# Autodesk Inventor assembly: map #2
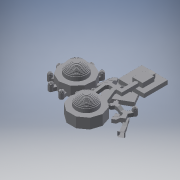
[picture p0: Inventor's stored thumbnail of the model, 180x180]
Saved by Autodesk Inventor 2017 (Build 210142000, 142)
## iProperties
Created: 2018-05-09
Part Number: map #2
Document SubType Name: Assembly
Designer: braxtonwright
Author: braxtonwright
## Documents named in this file (13)
- E:\School\Game develpment\geoscape\assembly\map #2.iam
- E:\School\Game develpment\geoscape\done\lowend map componts\corridors\corridor 2nd map.ipt
- E:\School\Game develpment\geoscape\done\lowend map componts\corridors\corridor 90 turn 2nd map.ipt
- E:\School\Game develpment\geoscape\done\lowend map componts\corridors\X corridor 2nd map.ipt
- E:\School\Game develpment\geoscape\done\lowend map componts\corridors\Y corridor 2nd map.ipt
- E:\School\Game develpment\geoscape\done\lowend map componts\rooms\starting room 2nd map.ipt
- E:\School\Game develpment\geoscape\done\lowend map componts\corridors\ramp 2nd map.ipt
- E:\School\Game develpment\geoscape\done\lowend map componts\rooms\room with 15 cubicals 2nd map.ipt
- E:\School\Game develpment\geoscape\done\lowend map componts\rooms\dome 2nd map.ipt
- E:\School\Game develpment\geoscape\done\lowend map componts\rooms\dome with corridors 2nd map.ipt
- E:\School\Game develpment\geoscape\done\lowend map componts\rooms\dome one terminal 2nd map.ipt
- E:\School\Game develpment\geoscape\rooms\(closed face) end door room (one wall) (9) 2nd map.ipt
- E:\School\Game develpment\geoscape\rooms\end door room (one wall) (9) 2nd map.ipt
## Components (56 placed, 12 different names)
1. corridor 2nd map:3 — Mate:91, Mate:92, Mate:97, Mate:98
2. ramp 2nd map:24 — Mate:89, Mate:90, Mate:91, Mate:92
3. ramp 2nd map:23 — Mate:85, Mate:86, Mate:87, Mate:88
4. ramp 2nd map:22 — Mate:81, Mate:82, Mate:83, Mate:84
5. ramp 2nd map:21 — Mate:77, Mate:78, Mate:79, Mate:80
6. corridor 90 turn 2nd map:9 — Mate:87, Mate:88, Mate:89, Mate:90
7. corridor 90 turn 2nd map:8 — Mate:83, Mate:84, Mate:85, Mate:86
8. corridor 90 turn 2nd map:7 — Mate:79, Mate:80, Mate:81, Mate:82
9. corridor 90 turn 2nd map:6 — Mate:77, Mate:78, Mate:93, Mate:94
10. Y corridor 2nd map:3 — Mate:73, Mate:74, Mate:75, Mate:76, Mate:93, Mate:94
11. ramp 2nd map:20 — Mate:71, Mate:72, Mate:73, Mate:74
12. Y corridor 2nd map:2 — Mate:67, Mate:68, Mate:69, Mate:70, Mate:71, Mate:72
13. ramp 2nd map:19 — Mate:61, Mate:62, Mate:67, Mate:68
14. ramp 2nd map:18 — Mate:60, Mate:61, Mate:62, Mate:63
15. ramp 2nd map:17 — Mate:59, Mate:60, Mate:63, Mate:64
16. ramp 2nd map:16 — Mate:59, Mate:64, Mate:65, Mate:66
17. corridor 90 turn 2nd map:5 — Mate:57, Mate:58, Mate:65, Mate:66
18. corridor 90 turn 2nd map:4 — Mate:55, Mate:56, Mate:57, Mate:58
19. ramp 2nd map:15 — Mate:31, Mate:34, Mate:35, Mate:36
20. ramp 2nd map:14 — Mate:30, Mate:31, Mate:33, Mate:34
21. ramp 2nd map:13 — Mate:29, Mate:30, Mate:32, Mate:33
22. corridor 2nd map:1 — Flush:1, Flush:5, Mate:1, Mate:5, Mate:6
23. corridor 2nd map:2 — Flush:1, Flush:2, Flush:5, Flush:6, Mate:1, Mate:2
24. corridor 90 turn 2nd map:2 — Flush:2, Flush:3, Flush:6, Flush:7, Mate:2, Mate:3
25. X corridor 2nd map:1 — Flush:3, Flush:4, Flush:7, Flush:8, Mate:3, Mate:4, Mate:7, Mate:10, Mate:19, Mate:22
26. Y corridor 2nd map:1 — Flush:4, Flush:8, Mate:4, Mate:8, Mate:9, Mate:20, Mate:21
27. ramp 2nd map:1 — Mate:9, Flush:17, Mate:15, Mate:20
28. ramp 2nd map:2 — Flush:19, Flush:20, Mate:17, Mate:18
29. ramp 2nd map:3 — Flush:20, Mate:18, Mate:25, Mate:26
30. ramp 2nd map:4 — Mate:10, Flush:19, Mate:17, Mate:19
31. ramp 2nd map:5 — Flush:17, Flush:18, Mate:15, Mate:16
32. ramp 2nd map:6 — Flush:18, Mate:16, Mate:55, Mate:56
33. ramp 2nd map:7 — Mate:8, Flush:15, Mate:13, Mate:21
34. ramp 2nd map:8 — Flush:15, Flush:16, Mate:13, Mate:14
35. ramp 2nd map:9 — Flush:16, Mate:14, Mate:27, Mate:28, Mate:29
36. ramp 2nd map:10 — Mate:7, Flush:13, Mate:11, Mate:22
37. ramp 2nd map:11 — Flush:13, Flush:14, Mate:11, Mate:12
38. ramp 2nd map:12 — Flush:14, Mate:12, Mate:23, Mate:24
39. dome 2nd map:1 — Mate:25, Mate:26
40. corridor 90 turn 2nd map:3 — Mate:27, Mate:28, Mate:32
41. (closed face) end door room (one wall) (9) 2nd map:1 — Mate:95, Mate:96
42. end door room (one wall) (9) 2nd map:1 — Mate:97, Mate:98
43. dome one terminal 2nd map:10 — Mate:75, Mate:76
44. room with 15 cubicals 2nd map:2 — Mate:69, Mate:70
45. dome with corridors 2nd map:1 — Mate:35, Mate:36, Mate:37, Mate:38, Mate:39, Mate:40, Mate:41, Mate:42, Mate:43, Mate:44, Mate:45, Mate:46, Mate:47, Mate:48, Mate:49, Mate:50, Mate:51, Mate:52, Mate:53, Mate:54
46. dome one terminal 2nd map:1 — Mate:37, Mate:54
47. dome one terminal 2nd map:2 — Mate:38, Mate:46
48. dome one terminal 2nd map:3 — Mate:39, Mate:47
49. dome one terminal 2nd map:4 — Mate:40, Mate:48
50. dome one terminal 2nd map:5 — Mate:41, Mate:49
51. dome one terminal 2nd map:6 — Mate:42, Mate:50
52. dome one terminal 2nd map:7 — Mate:43, Mate:51
53. dome one terminal 2nd map:8 — Mate:44, Mate:52
54. dome one terminal 2nd map:9 — Mate:45, Mate:53
55. starting room 2nd map:1 — Mate:5, Mate:6, Mate:95, Mate:96
56. room with 15 cubicals 2nd map:1 — Mate:23, Mate:24
## Relationships (114: Mate 98, Flush 16)
- Flush:1: corridor 2nd map:1 ↔ corridor 2nd map:2
- Flush:2: corridor 2nd map:2 ↔ corridor 90 turn 2nd map:2
- Flush:3: corridor 90 turn 2nd map:2 ↔ X corridor 2nd map:1
- Flush:4: X corridor 2nd map:1 ↔ Y corridor 2nd map:1
- Flush:5: corridor 2nd map:1 ↔ corridor 2nd map:2
- Flush:6: corridor 2nd map:2 ↔ corridor 90 turn 2nd map:2
- Flush:7: corridor 90 turn 2nd map:2 ↔ X corridor 2nd map:1
- Flush:8: X corridor 2nd map:1 ↔ Y corridor 2nd map:1
- Mate:1: corridor 2nd map:1 ↔ corridor 2nd map:2
- Mate:2: corridor 2nd map:2 ↔ corridor 90 turn 2nd map:2
- Mate:3: corridor 90 turn 2nd map:2 ↔ X corridor 2nd map:1
- Mate:4: X corridor 2nd map:1 ↔ Y corridor 2nd map:1
- Mate:5: corridor 2nd map:1 ↔ starting room 2nd map:1
- Mate:6: corridor 2nd map:1 ↔ starting room 2nd map:1
- Mate:7: X corridor 2nd map:1 ↔ ramp 2nd map:10
- Mate:8: Y corridor 2nd map:1 ↔ ramp 2nd map:7
- Mate:9: Y corridor 2nd map:1 ↔ ramp 2nd map:1
- Mate:10: X corridor 2nd map:1 ↔ ramp 2nd map:4
- Flush:13: ramp 2nd map:10 ↔ ramp 2nd map:11
- Flush:14: ramp 2nd map:11 ↔ ramp 2nd map:12
- Mate:11: ramp 2nd map:10 ↔ ramp 2nd map:11
- Mate:12: ramp 2nd map:11 ↔ ramp 2nd map:12
- Flush:15: ramp 2nd map:7 ↔ ramp 2nd map:8
- Flush:16: ramp 2nd map:8 ↔ ramp 2nd map:9
- Mate:13: ramp 2nd map:7 ↔ ramp 2nd map:8
- Mate:14: ramp 2nd map:8 ↔ ramp 2nd map:9
- Flush:17: ramp 2nd map:1 ↔ ramp 2nd map:5
- Flush:18: ramp 2nd map:5 ↔ ramp 2nd map:6
- Mate:15: ramp 2nd map:1 ↔ ramp 2nd map:5
- Mate:16: ramp 2nd map:5 ↔ ramp 2nd map:6
- Flush:19: ramp 2nd map:2 ↔ ramp 2nd map:4
- Flush:20: ramp 2nd map:2 ↔ ramp 2nd map:3
- Mate:17: ramp 2nd map:2 ↔ ramp 2nd map:4
- Mate:18: ramp 2nd map:2 ↔ ramp 2nd map:3
- Mate:19: X corridor 2nd map:1 ↔ ramp 2nd map:4
- Mate:20: Y corridor 2nd map:1 ↔ ramp 2nd map:1
- Mate:21: Y corridor 2nd map:1 ↔ ramp 2nd map:7
- Mate:22: X corridor 2nd map:1 ↔ ramp 2nd map:10
- Mate:23: ramp 2nd map:12 ↔ room with 15 cubicals 2nd map:1
- Mate:24: ramp 2nd map:12 ↔ room with 15 cubicals 2nd map:1
- Mate:25: ramp 2nd map:3 ↔ dome 2nd map:1
- Mate:26: ramp 2nd map:3 ↔ dome 2nd map:1
- Mate:27: ramp 2nd map:9 ↔ corridor 90 turn 2nd map:3
- Mate:28: ramp 2nd map:9 ↔ corridor 90 turn 2nd map:3
- Mate:29: ramp 2nd map:13 ↔ ramp 2nd map:9
- Mate:30: ramp 2nd map:14 ↔ ramp 2nd map:13
- Mate:31: ramp 2nd map:15 ↔ ramp 2nd map:14
- Mate:32: ramp 2nd map:13 ↔ corridor 90 turn 2nd map:3
- Mate:33: ramp 2nd map:14 ↔ ramp 2nd map:13
- Mate:34: ramp 2nd map:15 ↔ ramp 2nd map:14
- Mate:35: ramp 2nd map:15 ↔ dome with corridors 2nd map:1
- Mate:36: ramp 2nd map:15 ↔ dome with corridors 2nd map:1
- Mate:37: dome with corridors 2nd map:1 ↔ dome one terminal 2nd map:1
- Mate:38: dome with corridors 2nd map:1 ↔ dome one terminal 2nd map:2
- Mate:39: dome with corridors 2nd map:1 ↔ dome one terminal 2nd map:3
- Mate:40: dome with corridors 2nd map:1 ↔ dome one terminal 2nd map:4
- Mate:41: dome with corridors 2nd map:1 ↔ dome one terminal 2nd map:5
- Mate:42: dome with corridors 2nd map:1 ↔ dome one terminal 2nd map:6
- Mate:43: dome with corridors 2nd map:1 ↔ dome one terminal 2nd map:7
- Mate:44: dome with corridors 2nd map:1 ↔ dome one terminal 2nd map:8
- Mate:45: dome with corridors 2nd map:1 ↔ dome one terminal 2nd map:9
- Mate:46: dome with corridors 2nd map:1 ↔ dome one terminal 2nd map:2
- Mate:47: dome with corridors 2nd map:1 ↔ dome one terminal 2nd map:3
- Mate:48: dome with corridors 2nd map:1 ↔ dome one terminal 2nd map:4
- Mate:49: dome with corridors 2nd map:1 ↔ dome one terminal 2nd map:5
- Mate:50: dome with corridors 2nd map:1 ↔ dome one terminal 2nd map:6
- Mate:51: dome with corridors 2nd map:1 ↔ dome one terminal 2nd map:7
- Mate:52: dome with corridors 2nd map:1 ↔ dome one terminal 2nd map:8
- Mate:53: dome with corridors 2nd map:1 ↔ dome one terminal 2nd map:9
- Mate:54: dome with corridors 2nd map:1 ↔ dome one terminal 2nd map:1
- Mate:55: corridor 90 turn 2nd map:4 ↔ ramp 2nd map:6
- Mate:56: corridor 90 turn 2nd map:4 ↔ ramp 2nd map:6
- Mate:57: corridor 90 turn 2nd map:5 ↔ corridor 90 turn 2nd map:4
- Mate:58: corridor 90 turn 2nd map:5 ↔ corridor 90 turn 2nd map:4
- Mate:59: ramp 2nd map:17 ↔ ramp 2nd map:16
- Mate:60: ramp 2nd map:18 ↔ ramp 2nd map:17
- Mate:61: ramp 2nd map:19 ↔ ramp 2nd map:18
- Mate:62: ramp 2nd map:19 ↔ ramp 2nd map:18
- Mate:63: ramp 2nd map:18 ↔ ramp 2nd map:17
- Mate:64: ramp 2nd map:17 ↔ ramp 2nd map:16
- Mate:65: ramp 2nd map:16 ↔ corridor 90 turn 2nd map:5
- Mate:66: ramp 2nd map:16 ↔ corridor 90 turn 2nd map:5
- Mate:67: Y corridor 2nd map:2 ↔ ramp 2nd map:19
- Mate:68: Y corridor 2nd map:2 ↔ ramp 2nd map:19
- Mate:69: Y corridor 2nd map:2 ↔ room with 15 cubicals 2nd map:2
- Mate:70: Y corridor 2nd map:2 ↔ room with 15 cubicals 2nd map:2
- Mate:71: ramp 2nd map:20 ↔ Y corridor 2nd map:2
- Mate:72: ramp 2nd map:20 ↔ Y corridor 2nd map:2
- Mate:73: Y corridor 2nd map:3 ↔ ramp 2nd map:20
- Mate:74: Y corridor 2nd map:3 ↔ ramp 2nd map:20
- Mate:75: Y corridor 2nd map:3 ↔ dome one terminal 2nd map:10
- Mate:76: Y corridor 2nd map:3 ↔ dome one terminal 2nd map:10
- Mate:77: ramp 2nd map:21 ↔ corridor 90 turn 2nd map:6
- Mate:78: ramp 2nd map:21 ↔ corridor 90 turn 2nd map:6
- Mate:79: ramp 2nd map:21 ↔ corridor 90 turn 2nd map:7
- Mate:80: ramp 2nd map:21 ↔ corridor 90 turn 2nd map:7
- Mate:81: ramp 2nd map:22 ↔ corridor 90 turn 2nd map:7
- Mate:82: ramp 2nd map:22 ↔ corridor 90 turn 2nd map:7
- Mate:83: ramp 2nd map:22 ↔ corridor 90 turn 2nd map:8
- Mate:84: ramp 2nd map:22 ↔ corridor 90 turn 2nd map:8
- Mate:85: ramp 2nd map:23 ↔ corridor 90 turn 2nd map:8
- Mate:86: ramp 2nd map:23 ↔ corridor 90 turn 2nd map:8
- Mate:87: ramp 2nd map:23 ↔ corridor 90 turn 2nd map:9
- Mate:88: ramp 2nd map:23 ↔ corridor 90 turn 2nd map:9
- Mate:89: ramp 2nd map:24 ↔ corridor 90 turn 2nd map:9
- Mate:90: ramp 2nd map:24 ↔ corridor 90 turn 2nd map:9
- Mate:91: corridor 2nd map:3 ↔ ramp 2nd map:24
- Mate:92: corridor 2nd map:3 ↔ ramp 2nd map:24
- Mate:93: corridor 90 turn 2nd map:6 ↔ Y corridor 2nd map:3
- Mate:94: corridor 90 turn 2nd map:6 ↔ Y corridor 2nd map:3
- Mate:95: (closed face) end door room (one wall) (9) 2nd map:1 ↔ starting room 2nd map:1
- Mate:96: (closed face) end door room (one wall) (9) 2nd map:1 ↔ starting room 2nd map:1
- Mate:97: corridor 2nd map:3 ↔ end door room (one wall) (9) 2nd map:1
- Mate:98: corridor 2nd map:3 ↔ end door room (one wall) (9) 2nd map:1
